# Autodesk Inventor assembly: Antriebseinheit_ZSB
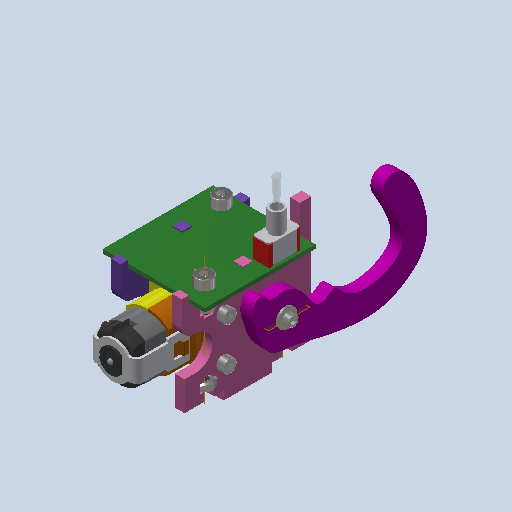
[picture p0: Inventor's stored thumbnail of the model, 512x512]
Saved by Autodesk Inventor 2025.2 (Build 292293000, 293)
## iProperties
Created: 2022-11-01
Part Number: Antriebseinheit_ZSB
Material: Generisch
Document SubType Name: Assembly
Designer: RP
Author: RP
## Documents named in this file (12)
- C:\Users\tino\Documents_VM\Konstruieren_CAD\Useless Box\_Useless_Box\Antriebseinheit_ZSB.iam
- C:\Users\tino\Documents_VM\Konstruieren_CAD\Useless Box\_Useless_Box\Motor_ZSB.iam
- C:\Users\tino\Documents_VM\Konstruieren_CAD\Useless Box\_Useless_Box\Motorhalter_rechts.ipt
- C:\Users\tino\Documents_VM\Konstruieren_CAD\Useless Box\_Useless_Box\Motorhalter_links.ipt
- C:\Users\tino\Documents_VM\Konstruieren_CAD\Useless Box\_Useless_Box\Finger.ipt
- C:\Users\tino\Documents_VM\Konstruieren_CAD\Useless Box\_Useless_Box\DIN 934 - M4 x 0,7.ipt
- C:\Users\tino\Documents_VM\Konstruieren_CAD\Useless Box\_Useless_Box\DIN EN ISO 4762 - M4 x 10.ipt
- C:\Users\tino\Documents_VM\Konstruieren_CAD\Useless Box\_Useless_Box\DIN EN ISO 4762 - M2,5 x 10.ipt
- C:\Users\tino\Documents_VM\Konstruieren_CAD\Useless Box\_Useless_Box\DIN 9021 - 2,7.ipt
- C:\Users\tino\Documents_VM\Konstruieren_CAD\Useless Box\_Useless_Box\DIN 934 - M3 x 0,5.ipt
- C:\Users\tino\Documents_VM\Konstruieren_CAD\Useless Box\_Useless_Box\DIN EN ISO 4762 - M3 x 30.ipt
- C:\Users\tino\Documents_VM\Konstruieren_CAD\Useless Box\_Useless_Box\Platine_ZSB.iam
## Components (19 placed, 11 different names)
1. Motor_ZSB:1 [sub-assembly] — Passend:20, Fluchtend:22, Passend:21, Winkel:8
2. Motorhalter_rechts:1
3. Motorhalter_links:1
4. Finger:1 — Winkel:8
5. DIN 934 - ersetzt durch DIN EN 24032/28673/28674 M4:1
6. DIN 934 - ersetzt durch DIN EN 24032/28673/28674 M4:2
7. DIN 934 - ersetzt durch DIN EN 24032/28673/28674 M4:3
8. DIN 934 - ersetzt durch DIN EN 24032/28673/28674 M4:4
9. DIN 934 - ersetzt durch DIN EN 24032/28673/28674 M4:5
10. DIN 934 - ersetzt durch DIN EN 24032/28673/28674 M4:6
11. DIN EN ISO 4762 M4 x 10:1
12. DIN EN ISO 4762 M2,5 x 10:1
13. DIN 9021 2,7:1
14. DIN 934 - ersetzt durch DIN EN 24032/28673/28674 M3:1
15. DIN EN ISO 4762 M3 x 30:1
16. DIN 934 - ersetzt durch DIN EN 24032/28673/28674 M3:2
17. DIN EN ISO 4762 M3 x 30:2
18. Platine_ZSB:1 [sub-assembly] — Einfügen:11
19. DIN EN ISO 4762 M4 x 10:2 — Einfügen:11
## Relationships (40: Mate 21, Insert 10, Angle 8, Flush 1)
- [Mate]: Motor_ZSB:1 ↔ Motorhalter_rechts:1
- [Mate]: Motor_ZSB:1 ↔ Motorhalter_links:1
- [Insert]: Motor_ZSB:1 ↔ Motorhalter_links:1
- [Insert]: Motor_ZSB:1 ↔ Motorhalter_rechts:1
- [Mate]: Motorhalter_links:1 ↔ Platine_ZSB:1
- [Mate]: Motorhalter_links:1 ↔ Platine_ZSB:1
- [Mate]: Motorhalter_rechts:1 ↔ Platine_ZSB:1
- [Mate]: Motor_ZSB:1 ↔ Finger:1
- [Mate]: Motor_ZSB:1 ↔ Finger:1
- [Mate]: Motorhalter_links:1 ↔ DIN 934 - ersetzt durch DIN EN 24032/28673/28674 M4:1
- [Angle] (0 deg): Motorhalter_links:1 ↔ DIN 934 - ersetzt durch DIN EN 24032/28673/28674 M4:1
- [Mate]: Motorhalter_links:1 ↔ DIN 934 - ersetzt durch DIN EN 24032/28673/28674 M4:1
- [Mate]: Motorhalter_links:1 ↔ DIN 934 - ersetzt durch DIN EN 24032/28673/28674 M4:2
- [Mate]: Motorhalter_links:1 ↔ DIN 934 - ersetzt durch DIN EN 24032/28673/28674 M4:2
- [Angle] (0 deg): Motorhalter_links:1 ↔ DIN 934 - ersetzt durch DIN EN 24032/28673/28674 M4:2
- [Mate]: Motorhalter_rechts:1 ↔ DIN 934 - ersetzt durch DIN EN 24032/28673/28674 M4:3
- [Mate]: Motorhalter_links:1 ↔ DIN 934 - ersetzt durch DIN EN 24032/28673/28674 M4:4
- [Mate]: Motorhalter_rechts:1 ↔ DIN 934 - ersetzt durch DIN EN 24032/28673/28674 M4:5
- [Mate]: Motorhalter_rechts:1 ↔ DIN 934 - ersetzt durch DIN EN 24032/28673/28674 M4:5
- [Mate]: Motorhalter_rechts:1 ↔ DIN 934 - ersetzt durch DIN EN 24032/28673/28674 M4:3
- [Mate]: Motorhalter_rechts:1 ↔ DIN 934 - ersetzt durch DIN EN 24032/28673/28674 M4:6
- [Mate]: Motorhalter_rechts:1 ↔ DIN 934 - ersetzt durch DIN EN 24032/28673/28674 M4:6
- [Angle] (0 deg): Motorhalter_rechts:1 ↔ DIN 934 - ersetzt durch DIN EN 24032/28673/28674 M4:6
- [Angle] (0 deg): Motorhalter_rechts:1 ↔ DIN 934 - ersetzt durch DIN EN 24032/28673/28674 M4:5
- [Angle] (0 deg): Motorhalter_links:1 ↔ DIN 934 - ersetzt durch DIN EN 24032/28673/28674 M4:4
- [Mate]: Motorhalter_links:1 ↔ DIN 934 - ersetzt durch DIN EN 24032/28673/28674 M4:4
- [Insert]: DIN EN ISO 4762 M4 x 10:1 ↔ Platine_ZSB:1
- [Insert]: Finger:1 ↔ DIN 9021 2,7:1
- [Insert]: DIN EN ISO 4762 M2,5 x 10:1 ↔ DIN 9021 2,7:1
- [Insert]: Motorhalter_links:1 ↔ DIN 934 - ersetzt durch DIN EN 24032/28673/28674 M3:1
- [Angle] (0 deg): Motorhalter_links:1 ↔ DIN 934 - ersetzt durch DIN EN 24032/28673/28674 M3:1
- [Insert]: Motorhalter_links:1 ↔ DIN 934 - ersetzt durch DIN EN 24032/28673/28674 M3:2
- [Angle] (0 deg): Motorhalter_links:1 ↔ DIN 934 - ersetzt durch DIN EN 24032/28673/28674 M3:2
- [Insert]: Motorhalter_rechts:1 ↔ DIN EN ISO 4762 M3 x 30:1
- [Insert]: Motorhalter_rechts:1 ↔ DIN EN ISO 4762 M3 x 30:2
- Passend:20 [Mate]: Motor_ZSB:1
- Fluchtend:22 [Flush]: Motor_ZSB:1
- Passend:21 [Mate]: Motor_ZSB:1
- Einfügen:11 [Insert]: Platine_ZSB:1 ↔ DIN EN ISO 4762 M4 x 10:2
- Winkel:8 [Angle] (180 deg): Motor_ZSB:1 ↔ Finger:1
